# Autodesk Inventor assembly: carriage
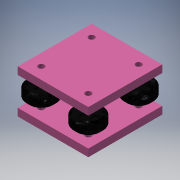
[picture p0: Inventor's stored thumbnail of the model, 180x180]
Saved by Autodesk Inventor 2019 (Build 230136000, 136)
## iProperties
Created: 2019-05-06
Part Number: carriage
Document SubType Name: Assembly
Designer: Alex Jones
Author: Alex Jones
## Documents named in this file (4)
- C:\Users\Alex Jones\Documents\Inventor\CNC\carriage.iam
- C:\Users\Alex Jones\Documents\Inventor\CNC\2020-1m.ipt
- C:\Users\Alex Jones\Documents\Inventor\CNC\roller.ipt
- C:\Users\Alex Jones\Documents\Inventor\CNC\CarriagePlate.ipt
## Components (7 placed, 3 different names)
1. 2020-1m:1 — Tangent:13, Tangent:14, Tangent:15, Tangent:16, Tangent:17, Tangent:18, Tangent:19, Tangent:20, Flush:1, Mate:28
2. roller:2 — Tangent:15, Tangent:16, Mate:16
3. roller:3 — Tangent:13, Tangent:14, Mate:17, Tangent:21
4. roller:5 — Tangent:19, Tangent:20, Mate:18
5. roller:6 — Tangent:17, Tangent:18, Mate:19, Mate:26
6. CarriagePlate:1 — Mate:27, Flush:2, Flush:3
7. CarriagePlate:2 — Mate:26, Mate:27, Mate:28, Flush:2, Flush:3, Tangent:21
## Relationships (25: Mate 13, Tangent 9, Flush 3)
- Tangent:13: 2020-1m:1 ↔ roller:3
- Tangent:14: 2020-1m:1 ↔ roller:3
- Tangent:15: 2020-1m:1 ↔ roller:2
- Tangent:16: 2020-1m:1 ↔ roller:2
- Tangent:17: 2020-1m:1 ↔ roller:6
- Tangent:18: 2020-1m:1 ↔ roller:6
- Tangent:19: 2020-1m:1 ↔ roller:5
- Tangent:20: 2020-1m:1 ↔ roller:5
- Mate:16: roller:2
- Mate:17: roller:3
- Mate:18: roller:5
- Mate:19: roller:6
- Mate:20
- Mate:21
- Mate:22
- Mate:23
- Mate:24
- Mate:25 (40 mm)
- Flush:1 (1.905 mm): 2020-1m:1
- Mate:26: roller:6 ↔ CarriagePlate:2
- Mate:27 (24.2 mm): CarriagePlate:1 ↔ CarriagePlate:2
- Mate:28 (2.1 mm): 2020-1m:1 ↔ CarriagePlate:2
- Flush:2: CarriagePlate:1 ↔ CarriagePlate:2
- Flush:3: CarriagePlate:1 ↔ CarriagePlate:2
- Tangent:21: roller:3 ↔ CarriagePlate:2
